# Autodesk Inventor assembly: 775pro_2_E_1-2inHex
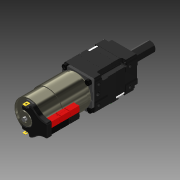
[picture p0: Inventor's stored thumbnail of the model, 180x180]
Saved by Autodesk Inventor 2022 (Build 260153000, 153)
## iProperties
Created: 2018-08-19
Part Number: 775pro_2_E_1-2inHex
Document SubType Name: Assembly
Mass: 1123.04 g
Surface Area: 1203.25 cm^2
Volume: 285.054 cm^3
Density: 3.93975 g/cm^3
## Documents named in this file (11)
- E:\Middleton Robotics\Collaborative Robots\Collaborative Part Library\General Gearboxes\Planetaries\Versaplanetary\VersaPlanetary\775pro, 2 Stages, Encoder, 1-2in Hex Output.iam
- E:\Middleton Robotics\Collaborative Robots\Collaborative Part Library\General Gearboxes\Planetaries\Versaplanetary\Intermediate Stages\Ring Gear.ipt
- E:\Middleton Robotics\Collaborative Robots\Collaborative Part Library\General Gearboxes\Planetaries\Versaplanetary\Intermediate Stages\VP Encoder.iam
- E:\Middleton Robotics\Collaborative Robots\Collaborative Part Library\General Gearboxes\Planetaries\Versaplanetary\V2 Stages\V2 Input Stage.iam
- E:\Middleton Robotics\Collaborative Robots\Collaborative Part Library\General Gearboxes\Planetaries\Versaplanetary\Screws\8-32 x 2.25in Screw.ipt
- E:\Middleton Robotics\Collaborative Robots\Collaborative Part Library\Power Transfer\Bearings and Bushings\Bearings\6902ZZ.ipt
- E:\Middleton Robotics\Collaborative Robots\Colaborative Part Library\General Gearboxes\Planetaries\Versaplanetary\V2 Stages\V2 Output Stage.iam
- E:\Middleton Robotics\Collaborative Robots\Collaborative Part Library\Power Transfer\Bearings.ipt
- E:\Middleton Robotics\Collaborative Robots\Collaborative Part Library\General Gearboxes\Planetaries\Versaplanetary\V2 Stages\V2 Output Stage\VP V2 Output Stage 1-2in Hex.iam
- E:\Middleton Robotics\Collaborative Robots\Collaborative Part Library\General Gearboxes\Planetaries\Versaplanetary\V2 Stages\V2 Input Stage\VP 775pro Input.iam
- E:\Middleton Robotics\Collaborative Robots\Collaborative Part Library\General Gearboxes\Planetaries\Versaplanetary\VersaPlanetary.iam
## Components (8 placed, 6 different names)
1. VP V2 Output Stage 1-2in Hex:1 [sub-assembly] — EncoderConstraint1, EncoderConstraint2, EncoderConstraint3, Flush:6, 2StageBasicInputMate2, Insert:25
2. Ring Gear 2 — Mate:4, Mate:5, Flush:6, 2StageBasicInputMate1
3. VP Encoder:1 [sub-assembly] — EncoderConstraint1, EncoderConstraint2, EncoderConstraint3, Mate:4, Mate:5
4. VP 775pro Input:1 [sub-assembly] — 2StageBasicInputMate1, 2StageBasicInputMate2, Insert:10, Insert:11
5. 8-32 x 2.25in Screw:1 — Insert:10
6. 8-32 x 2.25in Screw:2 — Insert:11
7. 6902ZZ:1
8. 6902ZZ:2 — Insert:25
## Relationships (11: Mate 4, Insert 4, Flush 2, Angle 1)
- EncoderConstraint1 [Mate]: VP V2 Output Stage 1-2in Hex:1 ↔ VP Encoder:1
- EncoderConstraint2 [Mate]: VP V2 Output Stage 1-2in Hex:1 ↔ VP Encoder:1
- EncoderConstraint3 [Angle] (0 deg): VP V2 Output Stage 1-2in Hex:1 ↔ VP Encoder:1
- Mate:4: Ring Gear 2 ↔ VP Encoder:1
- Mate:5: Ring Gear 2 ↔ VP Encoder:1
- Flush:6: VP V2 Output Stage 1-2in Hex:1 ↔ Ring Gear 2
- 2StageBasicInputMate1 [Insert]: Ring Gear 2 ↔ VP 775pro Input:1
- 2StageBasicInputMate2 [Flush]: VP V2 Output Stage 1-2in Hex:1 ↔ VP 775pro Input:1
- Insert:10: VP 775pro Input:1 ↔ 8-32 x 2.25in Screw:1
- Insert:11: VP 775pro Input:1 ↔ 8-32 x 2.25in Screw:2
- Insert:25: VP V2 Output Stage 1-2in Hex:1 ↔ 6902ZZ:2
